# Autodesk Inventor assembly: Water Table
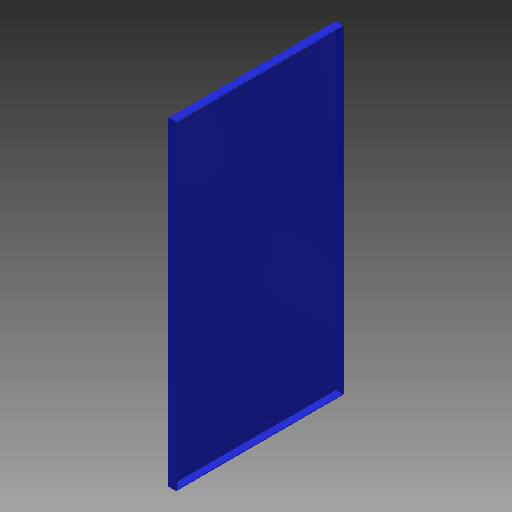
[picture p0: Inventor's stored thumbnail of the model, 512x512]
Saved by Autodesk Inventor 2018.2 (Build 222227000, 227)
## iProperties
Created: 2017-12-19
Part Number: Water Table
Document SubType Name: Assembly
Designer: torba
Author: torba
## Documents named in this file (5)
- C:\Users\torba\OneDrive\Documents\Inventor\Plasma 5x10\Water Table.iam
- C:\Users\torba\OneDrive\Documents\Inventor\Plasma 5x10\3 x 3 angle 45 .25 steel\3 x 3 angle 45 .25 steel-66.ipt
- C:\Users\torba\OneDrive\Documents\Inventor\Plasma 5x10\3 x 3 angle 45 .25 steel.ipt
- C:\Users\torba\OneDrive\Documents\Inventor\Plasma 5x10\3 x 3 angle 45 .25 steel\3 x 3 angle 45 .25 steel-126.ipt
- C:\Users\torba\OneDrive\Documents\Inventor\Plasma 5x10\1-16 sheet metal.ipt
## Components (5 placed, 3 different names)
1. 3 x 3 angle 45 .25 steel-126:1 — Flush:2, Mate:3, Mate:4, Flush:3, Mate:6
2. 3 x 3 angle 45 .25 steel-126:2 — Mate:1, Flush:1, Mate:2, Mate:5, Mate:7, Mate:8
3. 3 x 3 angle 45 .25 steel-66:3 — Mate:1, Flush:1, Mate:2, Flush:2, Mate:3, Mate:4, Mate:9
4. 3 x 3 angle 45 .25 steel-66:4 — Flush:3, Mate:5, Mate:6
5. 1-16 sheet metal:1 — Mate:7, Mate:8, Mate:9
## Relationships (12: Mate 9, Flush 3)
- Mate:1: 3 x 3 angle 45 .25 steel-126:2 ↔ 3 x 3 angle 45 .25 steel-66:3
- Flush:1: 3 x 3 angle 45 .25 steel-126:2 ↔ 3 x 3 angle 45 .25 steel-66:3
- Mate:2: 3 x 3 angle 45 .25 steel-126:2 ↔ 3 x 3 angle 45 .25 steel-66:3
- Flush:2: 3 x 3 angle 45 .25 steel-126:1 ↔ 3 x 3 angle 45 .25 steel-66:3
- Mate:3: 3 x 3 angle 45 .25 steel-126:1 ↔ 3 x 3 angle 45 .25 steel-66:3
- Mate:4: 3 x 3 angle 45 .25 steel-126:1 ↔ 3 x 3 angle 45 .25 steel-66:3
- Flush:3: 3 x 3 angle 45 .25 steel-126:1 ↔ 3 x 3 angle 45 .25 steel-66:4
- Mate:5: 3 x 3 angle 45 .25 steel-126:2 ↔ 3 x 3 angle 45 .25 steel-66:4
- Mate:6: 3 x 3 angle 45 .25 steel-126:1 ↔ 3 x 3 angle 45 .25 steel-66:4
- Mate:7: 3 x 3 angle 45 .25 steel-126:2 ↔ 1-16 sheet metal:1
- Mate:8: 3 x 3 angle 45 .25 steel-126:2 ↔ 1-16 sheet metal:1
- Mate:9: 3 x 3 angle 45 .25 steel-66:3 ↔ 1-16 sheet metal:1
